# Autodesk Inventor assembly: Head_Assembly
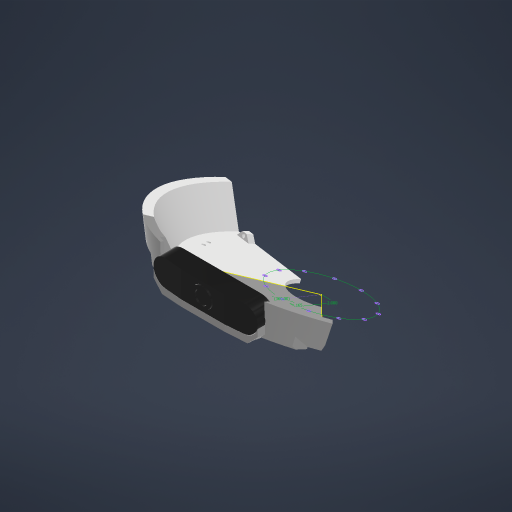
[picture p0: Inventor's stored thumbnail of the model, 512x512]
Saved by Autodesk Inventor 2024 (Build 280153000, 153)
## iProperties
Created: 2025-09-16
Part Number: Head_Assembly
Document SubType Name: Assembly
Designer: kevin
Author: kevin
## Documents named in this file (4)
- C:\Users\kevin\Desktop\SeniorDesign\Head_Assembly.iam
- C:\Users\kevin\Desktop\SeniorDesign\Emeet_Camera.ipt
- C:\Users\kevin\Desktop\SeniorDesign\Head_CameraPanel_Bottom.ipt
- C:\Users\kevin\Desktop\SeniorDesign\Head_BottomRight.ipt
## Components (3 placed, 3 different names)
1. Emeet_Camera:1 — Flush:1, Flush:2, Flush:3, Flush:4, Flush:5, Flush:6
2. Head_CameraPanel_Bottom:1 — Flush:1, Flush:2, Flush:3, Flush:4, Flush:5, Flush:6, Flush:7, Flush:8
3. Head_BottomRight:1 — Flush:7, Flush:8
## Relationships (8: Flush 8)
- Flush:1: Emeet_Camera:1 ↔ Head_CameraPanel_Bottom:1
- Flush:2 (0.2032 mm): Emeet_Camera:1 ↔ Head_CameraPanel_Bottom:1
- Flush:3 (0.508 mm): Emeet_Camera:1 ↔ Head_CameraPanel_Bottom:1
- Flush:4: Emeet_Camera:1 ↔ Head_CameraPanel_Bottom:1
- Flush:5: Emeet_Camera:1 ↔ Head_CameraPanel_Bottom:1
- Flush:6: Emeet_Camera:1 ↔ Head_CameraPanel_Bottom:1
- Flush:7: Head_CameraPanel_Bottom:1 ↔ Head_BottomRight:1
- Flush:8: Head_CameraPanel_Bottom:1 ↔ Head_BottomRight:1
